# Autodesk Inventor assembly: Intake Assembly
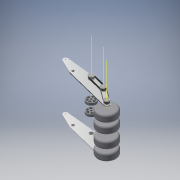
[picture p0: Inventor's stored thumbnail of the model, 180x180]
Saved by Autodesk Inventor 2019.4 (Build 234330000, 330)
## iProperties
Created: 2020-01-27
Part Number: Intake Assembly
Document SubType Name: Assembly
Designer: admin
Author: admin
## Documents named in this file (8)
- C:\Users\admin\Desktop\FRC 2020 Engineering\GitHub\7738-2020\Robot V2\Intake System\Intake Assembly.iam
- C:\Users\admin\Desktop\FRC 2020 Engineering\GitHub\7738-2020\Robot V2\Intake System\Intake Arm.ipt
- C:\Users\admin\Desktop\FRC 2020 Engineering\GitHub\7738-2020\Robot V2\Intake System\MF148ZZ.ipt
- C:\Users\admin\Desktop\FRC 2020 Engineering\GitHub\7738-2020\Robot V2\Turret\F6800.ipt
- C:\Users\admin\Desktop\FRC 2020 Engineering\GitHub\7738-2020\Robot V2\Intake System\2in Compliant Wheel.ipt
- C:\Users\admin\Desktop\FRC 2020 Engineering\GitHub\7738-2020\Robot V2\Intake System\Main Intake Wheel.ipt
- C:\Users\admin\Desktop\FRC 2020 Engineering\GitHub\7738-2020\Robot V2\Intake System\Intake Assembly\Design Accelerator\Synchronous Belts Transmission1.iam
- C:\Users\admin\Desktop\FRC 2020 Engineering\GitHub\7738-2020\Robot V2\Intake System\Intake Assembly\Design Accelerator\Synchronous Belts Transmission2.iam
## Components (20 placed, 6 different names)
1. Intake Arm:1 — Mate:1, Mate:2, Mate:3, Mate:4, Mate:7, Mate:8, Mate:12, Mate:15, Mate:16, Mate:17, Mate:18
2. Intake Arm:2 — Mate:1, Mate:2, Mate:5, Mate:6, Mate:9, Mate:10, Mate:12, Mate:13, Mate:14, Mate:19, Mate:20
3. MF148ZZ:2 — Mate:3, Mate:7, Mate:25
4. MF148ZZ:3 — Mate:4, Mate:8, Mate:11
5. MF148ZZ:4 — Mate:5, Mate:10
6. MF148ZZ:5 — Mate:6, Mate:9
7. F6800:1 — Mate:14, Mate:20, Mate:24
8. F6800:2 — Mate:13, Mate:19, Mate:21
9. F6800:3 — Mate:16, Mate:18, Mate:23
10. F6800:4 — Mate:15, Mate:17, Mate:22
11. 2in Compliant Wheel:1 — Mate:24, Flush:2
12. 2in Compliant Wheel:2 — Mate:21, Flush:2
13. 2in Compliant Wheel:3 — Mate:23, Flush:1
14. 2in Compliant Wheel:4 — Mate:22, Flush:1
15. Main Intake Wheel:1 — Mate:25, Mate:26, Mate:27
16. Main Intake Wheel:2 — Mate:26, Mate:28
17. Main Intake Wheel:3 — Mate:27
18. Main Intake Wheel:4 — Mate:28
19. Synchronous Belts Transmission:1 [sub-assembly]
20. Synchronous Belts Transmission:2 [sub-assembly]
## Relationships (30: Mate 28, Flush 2)
- Mate:1: Intake Arm:1 ↔ Intake Arm:2
- Mate:2: Intake Arm:1 ↔ Intake Arm:2
- Mate:3: Intake Arm:1 ↔ MF148ZZ:2
- Mate:4: Intake Arm:1 ↔ MF148ZZ:3
- Mate:5: Intake Arm:2 ↔ MF148ZZ:4
- Mate:6: Intake Arm:2 ↔ MF148ZZ:5
- Mate:7 (0.2 mm): Intake Arm:1 ↔ MF148ZZ:2
- Mate:8 (0.2 mm): Intake Arm:1 ↔ MF148ZZ:3
- Mate:9 (0.2 mm): Intake Arm:2 ↔ MF148ZZ:5
- Mate:10 (0.2 mm): Intake Arm:2 ↔ MF148ZZ:4
- Mate:11: MF148ZZ:3
- Mate:12 (248.6 mm): Intake Arm:1 ↔ Intake Arm:2
- Mate:13: Intake Arm:2 ↔ F6800:2
- Mate:14: Intake Arm:2 ↔ F6800:1
- Mate:15: Intake Arm:1 ↔ F6800:4
- Mate:16: Intake Arm:1 ↔ F6800:3
- Mate:17 (0.2 mm): Intake Arm:1 ↔ F6800:4
- Mate:18 (0.2 mm): Intake Arm:1 ↔ F6800:3
- Mate:19 (0.2 mm): Intake Arm:2 ↔ F6800:2
- Mate:20 (0.2 mm): Intake Arm:2 ↔ F6800:1
- Mate:21: F6800:2 ↔ 2in Compliant Wheel:2
- Mate:22: F6800:4 ↔ 2in Compliant Wheel:4
- Mate:23: F6800:3 ↔ 2in Compliant Wheel:3
- Mate:24: F6800:1 ↔ 2in Compliant Wheel:1
- Flush:1: 2in Compliant Wheel:3 ↔ 2in Compliant Wheel:4
- Flush:2: 2in Compliant Wheel:1 ↔ 2in Compliant Wheel:2
- Mate:25: MF148ZZ:2 ↔ Main Intake Wheel:1
- Mate:26: Main Intake Wheel:1 ↔ Main Intake Wheel:2
- Mate:27: Main Intake Wheel:1 ↔ Main Intake Wheel:3
- Mate:28: Main Intake Wheel:2 ↔ Main Intake Wheel:4
